# Autodesk Inventor assembly: 72. Шестерня второй передачи
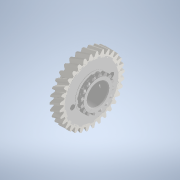
[picture p0: Inventor's stored thumbnail of the model, 180x180]
Saved by Autodesk Inventor 2021 (Build 250183000, 183)
## iProperties
Created: 2021-03-25
Part Number: 72. Шестерня второй передачи
Document SubType Name: Assembly
Designer: Данил
Author: Данил
## Documents named in this file (3)
- C:\Users\Данил\Desktop\Коробка передач\Детали\72. Шестерня второй передачи.iam
- C:\Users\Данил\Desktop\Коробка передач\Детали\72. Шестерня второй передачи.ipt
- C:\Users\Данил\Desktop\Коробка передач\Детали\72. Шестерня второй передачи\Мастер проектирования\Цилиндрическое зубчатое зацепление1.iam
## Components (2 placed, 2 different names)
1. 72. Шестерня второй передачи:1 — Совмещение:1, Заподлицо:1
2. Цилиндрическое зубчатое зацепление:1 [sub-assembly] — Совмещение:1, Заподлицо:1
## Relationships (2: Mate 1, Flush 1)
- Совмещение:1 [Mate]: 72. Шестерня второй передачи:1 ↔ Цилиндрическое зубчатое зацепление:1
- Заподлицо:1 [Flush]: 72. Шестерня второй передачи:1 ↔ Цилиндрическое зубчатое зацепление:1
